# Autodesk Inventor assembly: rail
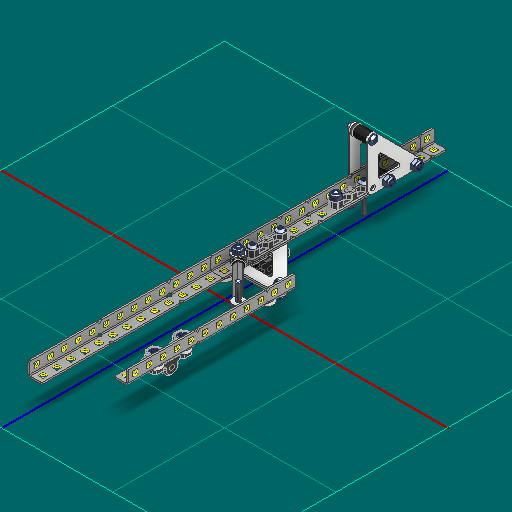
[picture p0: Inventor's stored thumbnail of the model, 512x512]
Saved by Autodesk Inventor 2025 (Build 290162000, 162)
## iProperties
Created: 2024-08-18
Part Number: rail
Document SubType Name: Assembly
Designer: averey
Author: averey
## Documents named in this file (26)
- C:\Users\avere\vex_robotics_high_stakes\hardware\cad\ATLAS\chassis\structure\rail.iam
- C:\Users\avere\vex_robotics_high_stakes\hardware\cad\ATLAS\chassis\structure\custom_parts\right_angle_gusset.ipt
- C:\Users\avere\vex_robotics_high_stakes\hardware\cad\VEX-CAD-Inventor\Structure\Hardware\Screw Shoulder Robosource\SScrew Shoulder Smooth .500 x .18.ipt
- C:\Users\avere\vex_robotics_high_stakes\hardware\cad\VEX-CAD-Inventor\Structure\Hardware\Screw Shoulder Robosource.ipt
- C:\Users\avere\vex_robotics_high_stakes\hardware\cad\VEX-CAD-Inventor\Structure\Hardware\Nut Thin Nylock.ipt
- C:\Users\avere\vex_robotics_high_stakes\hardware\cad\VEX-CAD-Inventor\Motion\Shaft LS\Bearing Flat Low Profile.ipt
- C:\Users\avere\vex_robotics_high_stakes\hardware\cad\VEX-CAD-Inventor\Structure\Hardware\Screw Steel - Star\SScrew Star Smooth 1.000.ipt
- C:\Users\avere\vex_robotics_high_stakes\hardware\cad\VEX-CAD-Inventor\Structure\Hardware\Screw Steel - Star.ipt
- C:\Users\avere\vex_robotics_high_stakes\hardware\cad\VEX-CAD-Inventor\Structure\Hardware\Screw Shoulder Robosource\SScrew Shoulder Smooth .500 x .04.ipt
- C:\Users\avere\vex_robotics_high_stakes\hardware\cad\VEX-CAD-Inventor\Structure\Angle\Aluminum 1x1\Alu Angle 1x1x28.ipt
- C:\Users\avere\vex_robotics_high_stakes\hardware\cad\VEX-CAD-Inventor\Structure\Angle\Aluminum 1x1\Alu Angle 1x1x15.ipt
- C:\Users\avere\vex_robotics_high_stakes\hardware\cad\ATLAS\chassis\structure\standoff_brace_triangle.iam
- C:\Users\avere\vex_robotics_high_stakes\hardware\cad\VEX-CAD-Inventor\Motion\Spacers\Spacer Nylon .500 OD\NSpacer White .500 OD x .125.ipt
- C:\Users\avere\vex_robotics_high_stakes\hardware\cad\VEX-CAD-Inventor\Motion\Spacers\Spacer Nylon .500 OD.ipt
- C:\Users\avere\vex_robotics_high_stakes\hardware\cad\VEX-CAD-Inventor\Structure\Hardware\Screw Steel - Star\SScrew Star Smooth .750.ipt
- C:\Users\avere\vex_robotics_high_stakes\hardware\cad\VEX-CAD-Inventor\Structure\Angle\Aluminum 1x1\Alu Angle 1x1x16.ipt
- C:\Users\avere\vex_robotics_high_stakes\hardware\cad\VEX-CAD-Inventor\Structure\Angle\Aluminum 1x1\Alu Angle 1x1x12.ipt
- C:\Users\avere\vex_robotics_high_stakes\hardware\cad\VEX-CAD-Inventor\Motion\Shaft LS\LS Pillow Bearing Block.ipt
- C:\Users\avere\vex_robotics_high_stakes\hardware\cad\_quick_assemblies\hex_nut_retainer_w_lock_nut.iam
- C:\Users\avere\vex_robotics_high_stakes\hardware\cad\VEX-CAD-Inventor\Structure\Hardware\Nut Nylon\Nut Nylon - White.ipt
- C:\Users\avere\vex_robotics_high_stakes\hardware\cad\VEX-CAD-Inventor\Structure\Hardware\Nut Nylon.ipt
- C:\Users\avere\vex_robotics_high_stakes\hardware\cad\VEX-CAD-Inventor\Motion\Spacers\Spacer Nylon .375 OD\NSpacer .375 OD x .125.ipt
- C:\Users\avere\vex_robotics_high_stakes\hardware\cad\VEX-CAD-Inventor\Motion\Spacers\Spacer Nylon .375 OD.ipt
- C:\Users\avere\vex_robotics_high_stakes\hardware\cad\VEX-CAD-Inventor\Motion\Spacers\Washer Steel\SWasher .375 OD x .062500.ipt
- C:\Users\avere\vex_robotics_high_stakes\hardware\cad\VEX-CAD-Inventor\Motion\Spacers\Washer Steel.ipt
- C:\Users\avere\vex_robotics_high_stakes\hardware\cad\ATLAS\tower\structure\triangle_brace.iam
## Components (37 placed, 19 different names)
1. right_angle_gusset:1 — Insert:19, Insert:30, Mate:13, Insert:38, Insert:39
2. right_angle_gusset:2 — Insert:1, Insert:21, Mate:15
3. SScrew Shoulder Smooth .500 x .18:1
4. Nut Thin Nylock:2 — Insert:1
5. Bearing Flat Low Profile:1
6. SScrew Star Smooth 1.000:1
7. SScrew Shoulder Smooth .500 x .04:3
8. Nut Thin Nylock:3
9. Alu Angle 1x1x28:1 — Mate:7
10. Alu Angle 1x1x15:1 — Mate:6, Angle:1, Mate:7, Angle:2, Insert:14, Insert:20
11. standoff_brace_triangle:1 [sub-assembly] — Insert:16, Mate:9
12. SScrew Star Smooth 1.000:2 — Insert:22
13. NSpacer White .500 OD x .125:1 — Insert:14
14. Nut Thin Nylock:4 — Insert:16
15. SScrew Star Smooth .750:3 — Insert:19
16. Alu Angle 1x1x16:1 — Insert:20, Insert:31, Mate:14, Mate:15, Insert:41, Mate:16, Insert:42
17. Alu Angle 1x1x12:1 — Insert:21, Insert:22, Mate:9, Insert:23, Mate:10, Insert:24, Insert:25, Insert:28, Mate:12, Insert:29, Insert:40
18. LS Pillow Bearing Block:1 — Insert:23, Mate:10, Insert:26, Insert:27
19. NSpacer White .500 OD x .125:2 — Insert:24
20. NSpacer White .500 OD x .125:3 — Insert:25, Mate:11
21. SScrew Shoulder Smooth .500 x .18:4 — Insert:26
22. SScrew Shoulder Smooth .500 x .18:5 — Insert:27
23. hex_nut_retainer_w_lock_nut:1 [sub-assembly] — Insert:28, Mate:11
24. hex_nut_retainer_w_lock_nut:2 [sub-assembly] — Mate:12, Insert:29
25. LS Pillow Bearing Block:2 — Insert:30, Mate:13, Insert:33, Insert:34
26. Bearing Flat Low Profile:2 — Insert:31, Mate:14, Insert:32, Insert:35
27. SScrew Star Smooth 1.000:4 — Insert:32
28. Nut Nylon - White:1 — Insert:33
29. SScrew Star Smooth 1.000:5 — Insert:35
30. Nut Nylon - White:2 — Insert:34
31. NSpacer .375 OD x .125:1 — Insert:36, Insert:39
32. SWasher .375 OD x .062500:1 — Insert:36
33. NSpacer .375 OD x .125:2 — Insert:38
34. SWasher .375 OD x .062500:2
35. NSpacer White .500 OD x .125:4 — Insert:40
36. triangle_brace:1 [sub-assembly] — Insert:41, Mate:16
37. Nut Thin Nylock:5 — Insert:42
## Relationships (50: Insert 34, Mate 14, Angle 2)
- Insert:1 (1.5875 mm): right_angle_gusset:2 ↔ Nut Thin Nylock:2
- [Insert] (1.27 mm): Bearing Flat Low Profile:1 ↔ SScrew Star Smooth 1.000:1
- [Insert] (1.27 mm): Bearing Flat Low Profile:1 ↔ Nut Thin Nylock:3
- [Mate]: right_angle_gusset:2 ↔ SScrew Shoulder Smooth .500 x .18:1
- [Insert] (1.5875 mm): Bearing Flat Low Profile:1 ↔ SScrew Shoulder Smooth .500 x .04:3
- [Insert]: Bearing Flat Low Profile:1 ↔ Alu Angle 1x1x28:1
- [Mate]: SScrew Star Smooth 1.000:1 ↔ Alu Angle 1x1x28:1
- [Mate]: right_angle_gusset:1 ↔ right_angle_gusset:2
- [Insert]: Alu Angle 1x1x15:1 ↔ standoff_brace_triangle:1
- [Mate]: right_angle_gusset:1 ↔ right_angle_gusset:2
- [Insert]: right_angle_gusset:2 ↔ Alu Angle 1x1x15:1
- [Insert] (1.5875 mm): right_angle_gusset:1 ↔ SScrew Shoulder Smooth .500 x .18:1
- Mate:6: Alu Angle 1x1x15:1
- Angle:1 (0 deg): Alu Angle 1x1x15:1
- Mate:7: Alu Angle 1x1x28:1 ↔ Alu Angle 1x1x15:1
- Angle:2 (0 deg): Alu Angle 1x1x15:1
- Insert:14: Alu Angle 1x1x15:1 ↔ NSpacer White .500 OD x .125:1
- Insert:16: standoff_brace_triangle:1 ↔ Nut Thin Nylock:4
- Insert:19 (1.5875 mm): right_angle_gusset:1 ↔ SScrew Star Smooth .750:3
- Insert:20: Alu Angle 1x1x15:1 ↔ Alu Angle 1x1x16:1
- Insert:21: right_angle_gusset:2 ↔ Alu Angle 1x1x12:1
- Insert:22: SScrew Star Smooth 1.000:2 ↔ Alu Angle 1x1x12:1
- Mate:9: standoff_brace_triangle:1 ↔ Alu Angle 1x1x12:1
- Insert:23 (3.175 mm): Alu Angle 1x1x12:1 ↔ LS Pillow Bearing Block:1
- Mate:10: Alu Angle 1x1x12:1 ↔ LS Pillow Bearing Block:1
- Insert:24: Alu Angle 1x1x12:1 ↔ NSpacer White .500 OD x .125:2
- Insert:25: Alu Angle 1x1x12:1 ↔ NSpacer White .500 OD x .125:3
- Insert:26: LS Pillow Bearing Block:1 ↔ SScrew Shoulder Smooth .500 x .18:4
- Insert:27: LS Pillow Bearing Block:1 ↔ SScrew Shoulder Smooth .500 x .18:5
- Insert:28: Alu Angle 1x1x12:1 ↔ hex_nut_retainer_w_lock_nut:1
- Mate:11: NSpacer White .500 OD x .125:3 ↔ hex_nut_retainer_w_lock_nut:1
- Mate:12: Alu Angle 1x1x12:1 ↔ hex_nut_retainer_w_lock_nut:2
- Insert:29: Alu Angle 1x1x12:1 ↔ hex_nut_retainer_w_lock_nut:2
- Insert:30 (4.7625 mm): right_angle_gusset:1 ↔ LS Pillow Bearing Block:2
- Mate:13: right_angle_gusset:1 ↔ LS Pillow Bearing Block:2
- Insert:31: Alu Angle 1x1x16:1 ↔ Bearing Flat Low Profile:2
- Mate:14: Alu Angle 1x1x16:1 ↔ Bearing Flat Low Profile:2
- Insert:32 (1.27 mm): Bearing Flat Low Profile:2 ↔ SScrew Star Smooth 1.000:4
- Insert:33: LS Pillow Bearing Block:2 ↔ Nut Nylon - White:1
- Insert:34: LS Pillow Bearing Block:2 ↔ Nut Nylon - White:2
- Insert:35 (1.27 mm): Bearing Flat Low Profile:2 ↔ SScrew Star Smooth 1.000:5
- Insert:36: NSpacer .375 OD x .125:1 ↔ SWasher .375 OD x .062500:1
- [Insert]: NSpacer .375 OD x .125:2 ↔ SWasher .375 OD x .062500:2
- Insert:38: right_angle_gusset:1 ↔ NSpacer .375 OD x .125:2
- Insert:39: right_angle_gusset:1 ↔ NSpacer .375 OD x .125:1
- Mate:15: right_angle_gusset:2 ↔ Alu Angle 1x1x16:1
- Insert:40: Alu Angle 1x1x12:1 ↔ NSpacer White .500 OD x .125:4
- Insert:41: Alu Angle 1x1x16:1 ↔ triangle_brace:1
- Mate:16: Alu Angle 1x1x16:1 ↔ triangle_brace:1
- Insert:42: Alu Angle 1x1x16:1 ↔ Nut Thin Nylock:5
## Named parameters: d76_d73 = 1.27 mm, d77_d75 = 1.27 mm, d60_d59 = 0 mm
